# Autodesk Inventor assembly: pol zaokraglona waska wysoka kwadraty
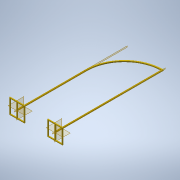
[picture p0: Inventor's stored thumbnail of the model, 180x180]
Saved by Autodesk Inventor 2021 (Build 250183000, 183)
## iProperties
Created: 2024-04-18
Part Number: pol zaokraglona waska wysoka kwadraty
Document SubType Name: Assembly
Designer: Michal
Author: Michal
## Documents named in this file (5)
- C:\Users\Michal\Documents\GitHub\PNW_PhotoBoothFrame_3D\pol zaokraglona waska wysoka kwadraty.iam
- C:\Users\Michal\Documents\GitHub\PNW_PhotoBoothFrame_3D\Stopa v1.iam
- C:\Users\Michal\Documents\GitHub\PNW_PhotoBoothFrame_3D\Lacznik prosty sruby.iam
- C:\Users\Michal\Documents\GitHub\PNW_PhotoBoothFrame_3D\Przedluzka L1500.ipt
- C:\Users\Michal\Documents\GitHub\PNW_PhotoBoothFrame_3D\pol luk R1000.ipt
## Components (7 placed, 4 different names)
1. Stopa v1:1 [sub-assembly] — Flush:1, Flush:2, Mate:40, Flush:8, Flush:9
2. Stopa v1:2 [sub-assembly] — Flush:1, Flush:2, Mate:41, Flush:10, Flush:11
3. Lacznik prosty sruby:1 [sub-assembly] — Flush:12, Mate:42, Mate:43, Mate:47, Mate:48, Mate:49
4. Przedluzka L1500:1 — Mate:40, Flush:8, Flush:9, Flush:12, Mate:42, Mate:43
5. Przedluzka L1500:2 — Mate:41, Flush:10, Flush:11, Mate:44, Mate:45, Mate:46
6. Lacznik prosty sruby:2 [sub-assembly] — Mate:44, Mate:45, Mate:46, Mate:50
7. pol luk R1000:1 — Mate:47, Mate:48, Mate:49, Mate:50
## Relationships (18: Mate 11, Flush 7)
- Flush:1: Stopa v1:1 ↔ Stopa v1:2
- Flush:2: Stopa v1:1 ↔ Stopa v1:2
- Mate:40: Stopa v1:1 ↔ Przedluzka L1500:1
- Flush:8: Stopa v1:1 ↔ Przedluzka L1500:1
- Flush:9: Stopa v1:1 ↔ Przedluzka L1500:1
- Mate:41: Stopa v1:2 ↔ Przedluzka L1500:2
- Flush:10: Stopa v1:2 ↔ Przedluzka L1500:2
- Flush:11: Stopa v1:2 ↔ Przedluzka L1500:2
- Flush:12: Lacznik prosty sruby:1 ↔ Przedluzka L1500:1
- Mate:42: Lacznik prosty sruby:1 ↔ Przedluzka L1500:1
- Mate:43: Lacznik prosty sruby:1 ↔ Przedluzka L1500:1
- Mate:44: Przedluzka L1500:2 ↔ Lacznik prosty sruby:2
- Mate:45: Przedluzka L1500:2 ↔ Lacznik prosty sruby:2
- Mate:46: Przedluzka L1500:2 ↔ Lacznik prosty sruby:2
- Mate:47: Lacznik prosty sruby:1 ↔ pol luk R1000:1
- Mate:48: Lacznik prosty sruby:1 ↔ pol luk R1000:1
- Mate:49: Lacznik prosty sruby:1 ↔ pol luk R1000:1
- Mate:50: Lacznik prosty sruby:2 ↔ pol luk R1000:1
